# Autodesk Inventor assembly: 9R015-57 Optikgruppe 429-III-SZ
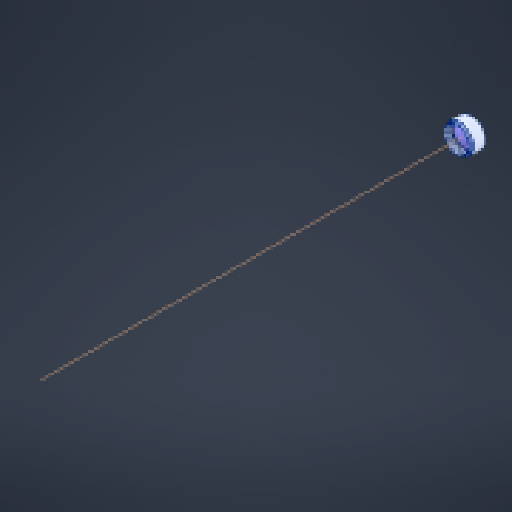
[picture p0: Inventor's stored thumbnail of the model, 512x512]
Saved by Autodesk Inventor 2025 (Build 290162000, 162)
## iProperties
Created: 2025-07-29
Part Number: 9R015-57 Optikgruppe 429-III-SZ
Document SubType Name: Assembly
Designer: mayhe
Author: mayhe
Revision Number: ANY
## Documents named in this file (4)
- C:\Users\mayhe\OneDrive\Documents\GitHub\In-situ-monitoring-of-powder-bed-fusion-additive-manufacturing\system_development\Adamant\v0.2\hardware_development\Cover parts\Xi-410-Camera-with-29°-x-18°-Lens\Xi 410 Camera with 29° x_2.iam
- C:\Users\mayhe\OneDrive\Documents\GitHub\In-situ-monitoring-of-powder-bed-fusion-additive-manufacturing\system_development\Adamant\v0.2\hardware_development\Cover parts\Xi-410-Camera-with-29°-x-18°-Lens\Xi 410 Camera with 29° x_8.ipt
- C:\Users\mayhe\OneDrive\Documents\GitHub\In-situ-monitoring-of-powder-bed-fusion-additive-manufacturing\system_development\Adamant\v0.2\hardware_development\Cover parts\Xi-410-Camera-with-29°-x-18°-Lens\Xi 410 Camera with 29° x_9.ipt
- C:\Users\mayhe\OneDrive\Documents\GitHub\In-situ-monitoring-of-powder-bed-fusion-additive-manufacturing\system_development\Adamant\v0.2\hardware_development\Cover parts\Xi-410-Camera-with-29°-x-18°-Lens\Xi 410 Camera with 29° x_10.ipt
## Components (3 placed, 3 different names)
1. 63118 O-Ring 18,5x1,5_8
2. 1R085-B Linse2-F13-384-GE-p17-RevB_9
3. 1R022-16 Frontschraubring-429-III_10 — Mate:1
## Relationships (1: Mate 1)
- Mate:1: 1R022-16 Frontschraubring-429-III_10
